# Autodesk Inventor assembly: kosi
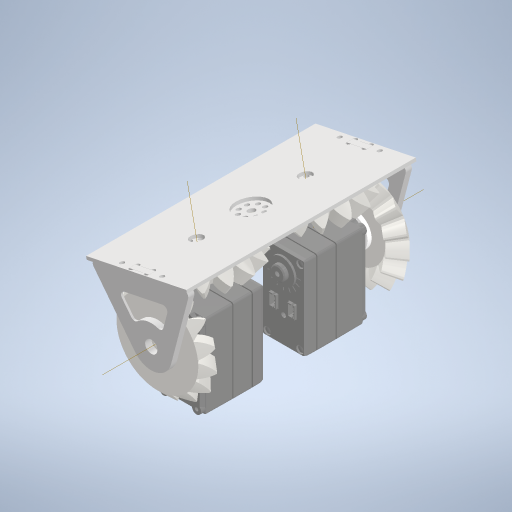
[picture p0: Inventor's stored thumbnail of the model, 512x512]
Saved by Autodesk Inventor 2024 (Build 280153000, 153)
## iProperties
Created: 2024-07-09
Part Number: kosi
Document SubType Name: Assembly
Designer: right
Author: right
## Documents named in this file (7)
- C:\Users\right\OneDrive\ドキュメント\Inventor\Vixen\kosi.iam
- C:\Users\right\OneDrive\ドキュメント\Inventor\Vixen\KRS2500_scale.ipt
- C:\Users\right\OneDrive\ドキュメント\Inventor\Vixen\kosi\デザイン アクセラレータ\かさ歯車1.iam
- C:\Users\right\OneDrive\ドキュメント\Inventor\Vixen\02157_SmallDiameterHornB.ipt
- C:\Users\right\OneDrive\ドキュメント\Inventor\Vixen\gia1.ipt
- C:\Users\right\OneDrive\ドキュメント\Inventor\Vixen\kosisita.ipt
- C:\Users\right\OneDrive\ドキュメント\Inventor\Vixen\kosipitch.ipt
## Components (12 placed, 6 different names)
1. かさ歯車:1 [sub-assembly] — 挿入:2, 挿入:3, 角度:1, 挿入:11, 角度:2, 挿入:15
2. KRS2500_scale:1 — 挿入:1, メイト:1, フラッシュ:1, フラッシュ:2
3. 02157_SmallDiameterHornB:1 — 挿入:1, 挿入:2, 挿入:3
4. かさ歯車:2 [sub-assembly] — 角度:1, 挿入:10, 挿入:12, 挿入:13, 挿入:14, 角度:4
5. KRS2500_scale:2 — メイト:1, フラッシュ:1, フラッシュ:2
6. 02157_SmallDiameterHornB:2
7. gia1:1 — 挿入:11, 角度:2
8. gia1:2 — 挿入:10, 挿入:12, 挿入:13
9. gia1:3 — 挿入:20
10. kosisita:1 — 角度:3, 挿入:16, 挿入:17, 挿入:18, 挿入:19, 角度:4, 挿入:20
11. kosipitch:1 — 挿入:14, 挿入:16, 挿入:17
12. kosipitch:2 — 挿入:15, 角度:3, 挿入:18, 挿入:19
## Relationships (24: Insert 17, Angle 4, Flush 2, Mate 1)
- 挿入:1 [Insert]: KRS2500_scale:1 ↔ 02157_SmallDiameterHornB:1
- 挿入:2 [Insert]: かさ歯車:1 ↔ 02157_SmallDiameterHornB:1
- 挿入:3 [Insert]: かさ歯車:1 ↔ 02157_SmallDiameterHornB:1
- [Insert]: KRS2500_scale:2 ↔ 02157_SmallDiameterHornB:2
- [Insert]: かさ歯車:2 ↔ 02157_SmallDiameterHornB:2
- [Insert]: かさ歯車:2 ↔ 02157_SmallDiameterHornB:2
- メイト:1 [Mate] (20 mm): KRS2500_scale:1 ↔ KRS2500_scale:2
- フラッシュ:1 [Flush]: KRS2500_scale:1 ↔ KRS2500_scale:2
- フラッシュ:2 [Flush]: KRS2500_scale:1 ↔ KRS2500_scale:2
- 角度:1 [Angle] (0 deg): かさ歯車:1 ↔ かさ歯車:2
- 挿入:10 [Insert]: かさ歯車:2 ↔ gia1:2
- 挿入:11 [Insert]: かさ歯車:1 ↔ gia1:1
- 角度:2 [Angle] (0 deg): かさ歯車:1 ↔ gia1:1
- 挿入:12 [Insert]: かさ歯車:2 ↔ gia1:2
- 挿入:13 [Insert]: かさ歯車:2 ↔ gia1:2
- 挿入:14 [Insert]: かさ歯車:2 ↔ kosipitch:1
- 挿入:15 [Insert]: かさ歯車:1 ↔ kosipitch:2
- 角度:3 [Angle] (0 deg): kosisita:1 ↔ kosipitch:2
- 挿入:16 [Insert]: kosisita:1 ↔ kosipitch:1
- 挿入:17 [Insert]: kosisita:1 ↔ kosipitch:1
- 挿入:18 [Insert]: kosisita:1 ↔ kosipitch:2
- 挿入:19 [Insert]: kosisita:1 ↔ kosipitch:2
- 角度:4 [Angle] (0 deg): かさ歯車:2 ↔ kosisita:1
- 挿入:20 [Insert]: gia1:3 ↔ kosisita:1
## Named parameters: d34_d32 = 0 mm, d35_d33 = 0 mm, d36_d31 = 0 mm
